# Autodesk Inventor assembly: Team_2374
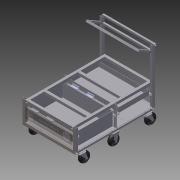
[picture p0: Inventor's stored thumbnail of the model, 180x180]
Saved by Autodesk Inventor 2012 (Build 160160000, 160)
## iProperties
Created: 2011-10-19
Part Number: Team_2374
Document SubType Name: Assembly
Designer: Ian Walters
Mass: 25411.4 g
Surface Area: 59424.9 cm^2
Volume: 9376.89 cm^3
Density: 2.71 g/cm^3
_SolveAssemblyDoc: Frame Generator Solve Assembly
_Version: 15.0.0
Author: Ian Walters
## Documents named in this file (38)
- C:\Users\Ian Walters\Dropbox\CAD Inventor\Preseason Projects\Cart Competition Cart\Team 2374\Team_2374.iam
- C:\Users\Ian Walters\Dropbox\CAD Inventor\Preseason Projects\Cart Competition Cart\Team 2374\Cart Skeleton.ipt
- C:\Users\Ian Walters\Dropbox\CAD Inventor\Preseason Projects\Cart Competition Cart\Team 2374\Team_2374\Frame\Cart Frame.iam
- C:\Users\Ian Walters\Dropbox\CAD Inventor\Preseason Projects\Cart Competition Cart\Team 2374\Bottom Sheet.ipt
- C:\Users\Ian Walters\Dropbox\CAD Inventor\Preseason Projects\Cart Competition Cart\Team 2374\IFI 114 - .1875 x 0.25.ipt
- C:\Users\Ian Walters\Dropbox\CAD Inventor\Preseason Projects\Cart Competition Cart\Team 2374\Fixed Caster.iam
- C:\Users\Ian Walters\Dropbox\CAD Inventor\Preseason Projects\Cart Competition Cart\Team 2374\Team_2374\Design Accelerator\Bolted Connection1.iam
- C:\Users\Ian Walters\Dropbox\CAD Inventor\Preseason Projects\Cart Competition Cart\Team 2374\Team_2374\Design Accelerator\Bolted Connection2.iam
- C:\Users\Ian Walters\Dropbox\CAD Inventor\Preseason Projects\Cart Competition Cart\Team 2374\Team_2374\Design Accelerator\Bolted Connection3.iam
- C:\Users\Ian Walters\Dropbox\CAD Inventor\Preseason Projects\Cart Competition Cart\Team 2374\Team_2374\Design Accelerator\Bolted Connection4.iam
- C:\Users\Ian Walters\Dropbox\CAD Inventor\Preseason Projects\Cart Competition Cart\Team 2374\Team_2374\Design Accelerator\Bolted Connection5.iam
- C:\Users\Ian Walters\Dropbox\CAD Inventor\Preseason Projects\Cart Competition Cart\Team 2374\Team_2374\Design Accelerator\Bolted Connection6.iam
- C:\Users\Ian Walters\Dropbox\CAD Inventor\Preseason Projects\Cart Competition Cart\Team 2374\Team_2374\Design Accelerator\Bolted Connection7.iam
- C:\Users\Ian Walters\Dropbox\CAD Inventor\Preseason Projects\Cart Competition Cart\Team 2374\Team_2374\Design Accelerator\Bolted Connection8.iam
- C:\Users\Ian Walters\Dropbox\CAD Inventor\Preseason Projects\Cart Competition Cart\Team 2374\Front Screen.ipt
- C:\Users\Ian Walters\Dropbox\CAD Inventor\Preseason Projects\Cart Competition Cart\Team 2374\Rotation Caster.iam
- C:\Users\Ian Walters\Dropbox\CAD Inventor\Preseason Projects\Cart Competition Cart\Team 2374\Team_2374\Design Accelerator\Bolted Connection9.iam
- C:\Users\Ian Walters\Dropbox\CAD Inventor\Preseason Projects\Cart Competition Cart\Team 2374\Team_2374\Design Accelerator\Bolted Connection10.iam
- C:\Users\Ian Walters\Dropbox\CAD Inventor\Preseason Projects\Cart Competition Cart\Team 2374\Team_2374\Design Accelerator\Bolted Connection11.iam
- C:\Users\Ian Walters\Dropbox\CAD Inventor\Preseason Projects\Cart Competition Cart\Team 2374\Team_2374\Design Accelerator\Bolted Connection12.iam
- C:\Users\Ian Walters\Dropbox\CAD Inventor\Preseason Projects\Cart Competition Cart\Team 2374\Team_2374\Design Accelerator\Bolted Connection13.iam
- C:\Users\Ian Walters\Dropbox\CAD Inventor\Preseason Projects\Cart Competition Cart\Team 2374\Team_2374\Design Accelerator\Bolted Connection14.iam
- C:\Users\Ian Walters\Dropbox\CAD Inventor\Preseason Projects\Cart Competition Cart\Team 2374\Team_2374\Design Accelerator\Bolted Connection15.iam
- C:\Users\Ian Walters\Dropbox\CAD Inventor\Preseason Projects\Cart Competition Cart\Team 2374\Team_2374\Design Accelerator\Bolted Connection16.iam
- C:\Users\Ian Walters\Dropbox\CAD Inventor\Preseason Projects\Cart Competition Cart\Team 2374\Team_2374\Design Accelerator\Bolted Connection17.iam
- C:\Users\Ian Walters\Dropbox\CAD Inventor\Preseason Projects\Cart Competition Cart\Team 2374\Team_2374\Design Accelerator\Bolted Connection18.iam
- C:\Users\Ian Walters\Dropbox\CAD Inventor\Preseason Projects\Cart Competition Cart\Team 2374\Team_2374\Design Accelerator\Bolted Connection19.iam
- C:\Users\Ian Walters\Dropbox\CAD Inventor\Preseason Projects\Cart Competition Cart\Team 2374\Team_2374\Design Accelerator\Bolted Connection20.iam
- C:\Users\Ian Walters\Dropbox\CAD Inventor\Preseason Projects\Cart Competition Cart\Team 2374\Team_2374\Design Accelerator\Bolted Connection21.iam
- C:\Users\Ian Walters\Dropbox\CAD Inventor\Preseason Projects\Cart Competition Cart\Team 2374\Team_2374\Design Accelerator\Bolted Connection22.iam
- C:\Users\Ian Walters\Dropbox\CAD Inventor\Preseason Projects\Cart Competition Cart\Team 2374\Team_2374\Design Accelerator\Bolted Connection23.iam
- C:\Users\Ian Walters\Dropbox\CAD Inventor\Preseason Projects\Cart Competition Cart\Team 2374\Team_2374\Design Accelerator\Bolted Connection24.iam
- C:\Users\Ian Walters\Dropbox\CAD Inventor\Preseason Projects\Cart Competition Cart\Team 2374\Drawer Slide.ipt
- C:\Users\Ian Walters\Dropbox\CAD Inventor\Preseason Projects\Cart Competition Cart\Team 2374\8020 Linear Bearing.iam
- C:\Users\Ian Walters\Dropbox\CAD Inventor\Preseason Projects\Cart Competition Cart\Team 2374\Big Drawer.ipt
- C:\Users\Ian Walters\Dropbox\CAD Inventor\Preseason Projects\Cart Competition Cart\Team 2374\Small Drawer.ipt
- C:\Users\Ian Walters\Dropbox\CAD Inventor\Preseason Projects\Cart Competition Cart\Team 2374\Handle.iam
- C:\Users\Ian Walters\Dropbox\CAD Inventor\Preseason Projects\Cart Competition Cart\Team 2374\Handle Slide.ipt
## Components (217 placed, 14 different names)
1. Cart Skeleton:1
2. Cart Frame:1 [sub-assembly] — Mate:1, Mate:2, Mate:3, Mate:4, Mate:5, Flush:1, Flush:2, Mate:26, Insert:11, Insert:12, Mate:29, Mate:30, Mate:31, Mate:32, Mate:33, Mate:34, Mate:35, Mate:36, Mate:37, Mate:38, Mate:39, Mate:40, Mate:41, Mate:42, Mate:43, Mate:44, Mate:45, Insert:13, Mate:46, Insert:14, Mate:47, Insert:15, Mate:48, Insert:16, Mate:49, Mate:50, Mate:51, Mate:52, Mate:53, Mate:54, Mate:55, Mate:56, Mate:57, Mate:58, Mate:59, Mate:60, Mate:61, Mate:62, Mate:63, Mate:64, Mate:65, Mate:66, Mate:67, Mate:68, Mate:69, Mate:70, Mate:71, Mate:72, Mate:73, Mate:74, Mate:75, Mate:76, Mate:77, Mate:78, Mate:79, Mate:80, Flush:3, Mate:81, Mate:83, Flush:21, Flush:22, Mate:92, Mate:93, Mate:94, Mate:95, Mate:96, Mate:99
3. Handle:1 [sub-assembly] — Mate:97, Mate:98, Mate:99
4. Handle Slide:2 — Mate:95, Mate:96, Flush:23
5. Handle Slide:1 — Mate:92, Mate:93, Mate:94, Flush:23, Mate:97, Mate:98
6. Bottom Sheet:1 — Mate:1, Mate:2, Mate:3, Insert:1, Insert:2, Insert:3, Insert:4, Mate:82
7. Front Screen:1 — Flush:1, Flush:2, Mate:26, Insert:7, Insert:8, Insert:9, Insert:10
8. Fixed Caster:1 [sub-assembly] — Mate:5, Insert:11
9. Fixed Caster:2 [sub-assembly] — Mate:4, Insert:12
10. Rotation Caster:1 [sub-assembly] — Mate:45, Insert:13
11. Rotation Caster:2 [sub-assembly] — Mate:46, Insert:14
12. Rotation Caster:3 [sub-assembly] — Mate:47, Insert:15
13. Rotation Caster:4 [sub-assembly] — Mate:48, Insert:16
14. IFI 114 - .1875 x 0.25:142 — Insert:10
15. IFI 114 - .1875 x 0.25:109 — Insert:7
16. Bolted Connection:1 [sub-assembly] — Mate:43, Mate:44
17. Bolted Connection:2 [sub-assembly] — Mate:29, Mate:30
18. Bolted Connection:3 [sub-assembly] — Mate:31, Mate:32
19. Bolted Connection:4 [sub-assembly] — Mate:33, Mate:34
20. Bolted Connection:5 [sub-assembly] — Mate:35, Mate:36
21. Bolted Connection:6 [sub-assembly] — Mate:37, Mate:38
22. Bolted Connection:7 [sub-assembly] — Mate:39, Mate:40
23. Bolted Connection:8 [sub-assembly] — Mate:41, Mate:42
24. Bolted Connection:9 [sub-assembly] — Mate:49, Mate:50
25. Bolted Connection:10 [sub-assembly] — Mate:51, Mate:52
26. Bolted Connection:11 [sub-assembly] — Mate:53, Mate:54
27. Bolted Connection:12 [sub-assembly] — Mate:55, Mate:56
28. Bolted Connection:13 [sub-assembly] — Mate:57, Mate:58
29. Bolted Connection:14 [sub-assembly] — Mate:59, Mate:60
30. Bolted Connection:15 [sub-assembly] — Mate:61, Mate:62
31. Bolted Connection:16 [sub-assembly] — Mate:63, Mate:64
32. Bolted Connection:17 [sub-assembly] — Mate:65, Mate:66
33. Bolted Connection:18 [sub-assembly] — Mate:67, Mate:68
34. Bolted Connection:19 [sub-assembly] — Mate:69, Mate:70
35. Bolted Connection:20 [sub-assembly] — Mate:71, Mate:72
36. Bolted Connection:21 [sub-assembly] — Mate:73, Mate:74
37. Bolted Connection:22 [sub-assembly] — Mate:75, Mate:76
38. Bolted Connection:23 [sub-assembly] — Mate:77, Mate:78
39. Bolted Connection:24 [sub-assembly] — Mate:79, Mate:80
40. Drawer Slide:1 — Flush:3, Mate:81, Mate:82, Flush:4, Flush:5, Flush:10, Flush:11, Flush:12, Flush:13
41. Drawer Slide:2 — Flush:4, Flush:5, Flush:9, Flush:16, Flush:17, Flush:18, Flush:19, Mate:89, Flush:8
42. Drawer Slide:3 — Flush:6, Flush:7, Flush:9, Mate:83, Mate:86, Flush:20, Mate:87, Mate:88
43. Drawer Slide:4 — Flush:6, Flush:7, Flush:8, Mate:84, Flush:14, Mate:85, Flush:15, Mate:89
44. 8020 Linear Bearing:1 [sub-assembly] — Flush:12, Flush:13, Insert:17, Insert:18
45. 8020 Linear Bearing:2 [sub-assembly] — Flush:10, Flush:11, Insert:19
46. 8020 Linear Bearing:3 [sub-assembly] — Mate:84, Flush:14, Insert:21
47. 8020 Linear Bearing:4 [sub-assembly] — Mate:85, Flush:15, Insert:20
48. 8020 Linear Bearing:5 [sub-assembly] — Flush:16, Flush:17, Mate:90
49. 8020 Linear Bearing:6 [sub-assembly] — Flush:18, Flush:19, Mate:91
50. 8020 Linear Bearing:7 [sub-assembly] — Mate:86, Flush:20, Insert:24
51. 8020 Linear Bearing:8 [sub-assembly] — Mate:87, Mate:88, Insert:22, Insert:23
52. Big Drawer:1 — Insert:17, Insert:18, Insert:19, Insert:20, Insert:21, Flush:21
53. Small Drawer:1 — Insert:22, Insert:23, Insert:24, Mate:90, Mate:91, Flush:22
54. IFI 114 - .1875 x 0.25:1 — Insert:1
55. IFI 114 - .1875 x 0.25:2 — Insert:2
56. IFI 114 - .1875 x 0.25:3 — Insert:3
57. IFI 114 - .1875 x 0.25:4 — Insert:4
58. IFI 114 - .1875 x 0.25:5
59. IFI 114 - .1875 x 0.25:6
60. IFI 114 - .1875 x 0.25:7
61. IFI 114 - .1875 x 0.25:8
62. IFI 114 - .1875 x 0.25:9
63. IFI 114 - .1875 x 0.25:10
64. IFI 114 - .1875 x 0.25:11
65. IFI 114 - .1875 x 0.25:12
66. IFI 114 - .1875 x 0.25:13
67. IFI 114 - .1875 x 0.25:14
68. IFI 114 - .1875 x 0.25:15
69. IFI 114 - .1875 x 0.25:16
70. IFI 114 - .1875 x 0.25:17
71. IFI 114 - .1875 x 0.25:18
72. IFI 114 - .1875 x 0.25:19
73. IFI 114 - .1875 x 0.25:20
74. IFI 114 - .1875 x 0.25:21
75. IFI 114 - .1875 x 0.25:22
76. IFI 114 - .1875 x 0.25:23
77. IFI 114 - .1875 x 0.25:24
78. IFI 114 - .1875 x 0.25:25
79. IFI 114 - .1875 x 0.25:26
80. IFI 114 - .1875 x 0.25:27
81. IFI 114 - .1875 x 0.25:28
82. IFI 114 - .1875 x 0.25:29
83. IFI 114 - .1875 x 0.25:30
84. IFI 114 - .1875 x 0.25:31
85. IFI 114 - .1875 x 0.25:32
86. IFI 114 - .1875 x 0.25:33
87. IFI 114 - .1875 x 0.25:34
88. IFI 114 - .1875 x 0.25:35
89. IFI 114 - .1875 x 0.25:36
90. IFI 114 - .1875 x 0.25:37
91. IFI 114 - .1875 x 0.25:38
92. IFI 114 - .1875 x 0.25:39
93. IFI 114 - .1875 x 0.25:40
94. IFI 114 - .1875 x 0.25:41
95. IFI 114 - .1875 x 0.25:42
96. IFI 114 - .1875 x 0.25:43
97. IFI 114 - .1875 x 0.25:44
98. IFI 114 - .1875 x 0.25:45
99. IFI 114 - .1875 x 0.25:46
100. IFI 114 - .1875 x 0.25:47
101. IFI 114 - .1875 x 0.25:48
102. IFI 114 - .1875 x 0.25:49
103. IFI 114 - .1875 x 0.25:50
104. IFI 114 - .1875 x 0.25:51
105. IFI 114 - .1875 x 0.25:52
106. IFI 114 - .1875 x 0.25:53
107. IFI 114 - .1875 x 0.25:54
108. IFI 114 - .1875 x 0.25:55
109. IFI 114 - .1875 x 0.25:56
110. IFI 114 - .1875 x 0.25:57
111. IFI 114 - .1875 x 0.25:58
112. IFI 114 - .1875 x 0.25:59
113. IFI 114 - .1875 x 0.25:60
114. IFI 114 - .1875 x 0.25:61
115. IFI 114 - .1875 x 0.25:62
116. IFI 114 - .1875 x 0.25:63
117. IFI 114 - .1875 x 0.25:64
118. IFI 114 - .1875 x 0.25:65
119. IFI 114 - .1875 x 0.25:66
120. IFI 114 - .1875 x 0.25:67
121. IFI 114 - .1875 x 0.25:68
122. IFI 114 - .1875 x 0.25:69
123. IFI 114 - .1875 x 0.25:70
124. IFI 114 - .1875 x 0.25:71
125. IFI 114 - .1875 x 0.25:72
126. IFI 114 - .1875 x 0.25:73
127. IFI 114 - .1875 x 0.25:74
128. IFI 114 - .1875 x 0.25:75
129. IFI 114 - .1875 x 0.25:76
130. IFI 114 - .1875 x 0.25:77
131. IFI 114 - .1875 x 0.25:78
132. IFI 114 - .1875 x 0.25:79
133. IFI 114 - .1875 x 0.25:80
134. IFI 114 - .1875 x 0.25:81
135. IFI 114 - .1875 x 0.25:82
136. IFI 114 - .1875 x 0.25:83
137. IFI 114 - .1875 x 0.25:84
138. IFI 114 - .1875 x 0.25:85
139. IFI 114 - .1875 x 0.25:86
140. IFI 114 - .1875 x 0.25:87
141. IFI 114 - .1875 x 0.25:88
142. IFI 114 - .1875 x 0.25:89
143. IFI 114 - .1875 x 0.25:90
144. IFI 114 - .1875 x 0.25:91
145. IFI 114 - .1875 x 0.25:92
146. IFI 114 - .1875 x 0.25:93
147. IFI 114 - .1875 x 0.25:94
148. IFI 114 - .1875 x 0.25:95
149. IFI 114 - .1875 x 0.25:96
150. IFI 114 - .1875 x 0.25:97
151. IFI 114 - .1875 x 0.25:98
152. IFI 114 - .1875 x 0.25:99
153. IFI 114 - .1875 x 0.25:100
154. IFI 114 - .1875 x 0.25:101
155. IFI 114 - .1875 x 0.25:102
156. IFI 114 - .1875 x 0.25:103
157. IFI 114 - .1875 x 0.25:104
158. IFI 114 - .1875 x 0.25:105
159. IFI 114 - .1875 x 0.25:106
160. IFI 114 - .1875 x 0.25:107
161. IFI 114 - .1875 x 0.25:108
162. IFI 114 - .1875 x 0.25:110 — Insert:8
163. IFI 114 - .1875 x 0.25:111
164. IFI 114 - .1875 x 0.25:112
165. IFI 114 - .1875 x 0.25:113
166. IFI 114 - .1875 x 0.25:114
167. IFI 114 - .1875 x 0.25:115
168. IFI 114 - .1875 x 0.25:116
169. IFI 114 - .1875 x 0.25:117
170. IFI 114 - .1875 x 0.25:118
171. IFI 114 - .1875 x 0.25:119
172. IFI 114 - .1875 x 0.25:120
173. IFI 114 - .1875 x 0.25:121
174. IFI 114 - .1875 x 0.25:122
175. IFI 114 - .1875 x 0.25:123
176. IFI 114 - .1875 x 0.25:124
177. IFI 114 - .1875 x 0.25:125
178. IFI 114 - .1875 x 0.25:126
179. IFI 114 - .1875 x 0.25:127
180. IFI 114 - .1875 x 0.25:128
181. IFI 114 - .1875 x 0.25:129
182. IFI 114 - .1875 x 0.25:130
183. IFI 114 - .1875 x 0.25:131
184. IFI 114 - .1875 x 0.25:132
185. IFI 114 - .1875 x 0.25:133
186. IFI 114 - .1875 x 0.25:134
187. IFI 114 - .1875 x 0.25:135
188. IFI 114 - .1875 x 0.25:136
189. IFI 114 - .1875 x 0.25:137
190. IFI 114 - .1875 x 0.25:138
191. IFI 114 - .1875 x 0.25:139
192. IFI 114 - .1875 x 0.25:140
193. IFI 114 - .1875 x 0.25:141 — Insert:9
194. IFI 114 - .1875 x 0.25:143
195. IFI 114 - .1875 x 0.25:144
196. IFI 114 - .1875 x 0.25:145
197. IFI 114 - .1875 x 0.25:146
198. IFI 114 - .1875 x 0.25:147
199. IFI 114 - .1875 x 0.25:148
200. IFI 114 - .1875 x 0.25:149
201. IFI 114 - .1875 x 0.25:150
202. IFI 114 - .1875 x 0.25:151
203. IFI 114 - .1875 x 0.25:152
204. IFI 114 - .1875 x 0.25:153
205. IFI 114 - .1875 x 0.25:154
206. IFI 114 - .1875 x 0.25:155
207. IFI 114 - .1875 x 0.25:156
208. IFI 114 - .1875 x 0.25:157
209. IFI 114 - .1875 x 0.25:158
210. IFI 114 - .1875 x 0.25:159
211. IFI 114 - .1875 x 0.25:160
212. IFI 114 - .1875 x 0.25:161
213. IFI 114 - .1875 x 0.25:162
214. IFI 114 - .1875 x 0.25:163
215. IFI 114 - .1875 x 0.25:164
216. IFI 114 - .1875 x 0.25:165
217. IFI 114 - .1875 x 0.25:166
## Component patterns: (27 elements, first: IFI 114 - .1875 x 0.25:1 + IFI 114 - .1875 x 0.25:2 + IFI 114 - .1875 x 0.25:3 + IFI 114 - .1875 x 0.25:4), (31 elements, first: IFI 114 - .1875 x 0.25:110), (25 elements, first: IFI 114 - .1875 x 0.25:141)
## Relationships (122: Mate 77, Flush 23, Insert 22)
- Mate:1: Cart Frame:1 ↔ Bottom Sheet:1
- Mate:2: Cart Frame:1 ↔ Bottom Sheet:1
- Mate:3: Cart Frame:1 ↔ Bottom Sheet:1
- Insert:1: Bottom Sheet:1 ↔ IFI 114 - .1875 x 0.25:1
- Insert:2: Bottom Sheet:1 ↔ IFI 114 - .1875 x 0.25:2
- Insert:3: Bottom Sheet:1 ↔ IFI 114 - .1875 x 0.25:3
- Insert:4: Bottom Sheet:1 ↔ IFI 114 - .1875 x 0.25:4
- Mate:4: Cart Frame:1 ↔ Fixed Caster:2
- Mate:5: Cart Frame:1 ↔ Fixed Caster:1
- Flush:1: Cart Frame:1 ↔ Front Screen:1
- Flush:2: Cart Frame:1 ↔ Front Screen:1
- Mate:26: Cart Frame:1 ↔ Front Screen:1
- Insert:7: Front Screen:1 ↔ IFI 114 - .1875 x 0.25:109
- Insert:8: Front Screen:1 ↔ IFI 114 - .1875 x 0.25:110
- Insert:9: Front Screen:1 ↔ IFI 114 - .1875 x 0.25:141
- Insert:10: Front Screen:1 ↔ IFI 114 - .1875 x 0.25:142
- Insert:11: Cart Frame:1 ↔ Fixed Caster:1
- Insert:12: Cart Frame:1 ↔ Fixed Caster:2
- Mate:29: Cart Frame:1 ↔ Bolted Connection:2
- Mate:30: Cart Frame:1 ↔ Bolted Connection:2
- Mate:31: Cart Frame:1 ↔ Bolted Connection:3
- Mate:32: Cart Frame:1 ↔ Bolted Connection:3
- Mate:33: Cart Frame:1 ↔ Bolted Connection:4
- Mate:34: Cart Frame:1 ↔ Bolted Connection:4
- Mate:35: Cart Frame:1 ↔ Bolted Connection:5
- Mate:36: Cart Frame:1 ↔ Bolted Connection:5
- Mate:37: Cart Frame:1 ↔ Bolted Connection:6
- Mate:38: Cart Frame:1 ↔ Bolted Connection:6
- Mate:39: Cart Frame:1 ↔ Bolted Connection:7
- Mate:40: Cart Frame:1 ↔ Bolted Connection:7
- Mate:41: Cart Frame:1 ↔ Bolted Connection:8
- Mate:42: Cart Frame:1 ↔ Bolted Connection:8
- Mate:43: Cart Frame:1 ↔ Bolted Connection:1
- Mate:44: Cart Frame:1 ↔ Bolted Connection:1
- Mate:45: Cart Frame:1 ↔ Rotation Caster:1
- Insert:13: Cart Frame:1 ↔ Rotation Caster:1
- Mate:46: Cart Frame:1 ↔ Rotation Caster:2
- Insert:14: Cart Frame:1 ↔ Rotation Caster:2
- Mate:47: Cart Frame:1 ↔ Rotation Caster:3
- Insert:15: Cart Frame:1 ↔ Rotation Caster:3
- Mate:48: Cart Frame:1 ↔ Rotation Caster:4
- Insert:16: Cart Frame:1 ↔ Rotation Caster:4
- Mate:49: Cart Frame:1 ↔ Bolted Connection:9
- Mate:50: Cart Frame:1 ↔ Bolted Connection:9
- Mate:51: Cart Frame:1 ↔ Bolted Connection:10
- Mate:52: Cart Frame:1 ↔ Bolted Connection:10
- Mate:53: Cart Frame:1 ↔ Bolted Connection:11
- Mate:54: Cart Frame:1 ↔ Bolted Connection:11
- Mate:55: Cart Frame:1 ↔ Bolted Connection:12
- Mate:56: Cart Frame:1 ↔ Bolted Connection:12
- Mate:57: Cart Frame:1 ↔ Bolted Connection:13
- Mate:58: Cart Frame:1 ↔ Bolted Connection:13
- Mate:59: Cart Frame:1 ↔ Bolted Connection:14
- Mate:60: Cart Frame:1 ↔ Bolted Connection:14
- Mate:61: Cart Frame:1 ↔ Bolted Connection:15
- Mate:62: Cart Frame:1 ↔ Bolted Connection:15
- Mate:63: Cart Frame:1 ↔ Bolted Connection:16
- Mate:64: Cart Frame:1 ↔ Bolted Connection:16
- Mate:65: Cart Frame:1 ↔ Bolted Connection:17
- Mate:66: Cart Frame:1 ↔ Bolted Connection:17
- Mate:67: Cart Frame:1 ↔ Bolted Connection:18
- Mate:68: Cart Frame:1 ↔ Bolted Connection:18
- Mate:69: Cart Frame:1 ↔ Bolted Connection:19
- Mate:70: Cart Frame:1 ↔ Bolted Connection:19
- Mate:71: Cart Frame:1 ↔ Bolted Connection:20
- Mate:72: Cart Frame:1 ↔ Bolted Connection:20
- Mate:73: Cart Frame:1 ↔ Bolted Connection:21
- Mate:74: Cart Frame:1 ↔ Bolted Connection:21
- Mate:75: Cart Frame:1 ↔ Bolted Connection:22
- Mate:76: Cart Frame:1 ↔ Bolted Connection:22
- Mate:77: Cart Frame:1 ↔ Bolted Connection:23
- Mate:78: Cart Frame:1 ↔ Bolted Connection:23
- Mate:79: Cart Frame:1 ↔ Bolted Connection:24
- Mate:80: Cart Frame:1 ↔ Bolted Connection:24
- Flush:3: Cart Frame:1 ↔ Drawer Slide:1
- Mate:81: Cart Frame:1 ↔ Drawer Slide:1
- Mate:82 (152.4 mm): Bottom Sheet:1 ↔ Drawer Slide:1
- Flush:4: Drawer Slide:1 ↔ Drawer Slide:2
- Flush:5: Drawer Slide:1 ↔ Drawer Slide:2
- Flush:6: Drawer Slide:3 ↔ Drawer Slide:4
- Flush:7: Drawer Slide:3 ↔ Drawer Slide:4
- Flush:8: Drawer Slide:2 ↔ Drawer Slide:4
- Flush:9: Drawer Slide:2 ↔ Drawer Slide:3
- Mate:83: Cart Frame:1 ↔ Drawer Slide:3
- Flush:10: Drawer Slide:1 ↔ 8020 Linear Bearing:2
- Flush:11: Drawer Slide:1 ↔ 8020 Linear Bearing:2
- Flush:12: Drawer Slide:1 ↔ 8020 Linear Bearing:1
- Flush:13: Drawer Slide:1 ↔ 8020 Linear Bearing:1
- Mate:84: Drawer Slide:4 ↔ 8020 Linear Bearing:3
- Flush:14: Drawer Slide:4 ↔ 8020 Linear Bearing:3
- Mate:85: Drawer Slide:4 ↔ 8020 Linear Bearing:4
- Flush:15: Drawer Slide:4 ↔ 8020 Linear Bearing:4
- Flush:16: Drawer Slide:2 ↔ 8020 Linear Bearing:5
- Flush:17: Drawer Slide:2 ↔ 8020 Linear Bearing:5
- Flush:18: Drawer Slide:2 ↔ 8020 Linear Bearing:6
- Flush:19: Drawer Slide:2 ↔ 8020 Linear Bearing:6
- Mate:86: Drawer Slide:3 ↔ 8020 Linear Bearing:7
- Flush:20: Drawer Slide:3 ↔ 8020 Linear Bearing:7
- Mate:87: Drawer Slide:3 ↔ 8020 Linear Bearing:8
- Mate:88: Drawer Slide:3 ↔ 8020 Linear Bearing:8
- Insert:17: 8020 Linear Bearing:1 ↔ Big Drawer:1
- Insert:18: 8020 Linear Bearing:1 ↔ Big Drawer:1
- Insert:19: 8020 Linear Bearing:2 ↔ Big Drawer:1
- Insert:20: 8020 Linear Bearing:4 ↔ Big Drawer:1
- Insert:21: 8020 Linear Bearing:3 ↔ Big Drawer:1
- Flush:21: Cart Frame:1 ↔ Big Drawer:1
- Mate:89 (25.4 mm): Drawer Slide:2 ↔ Drawer Slide:4
- Insert:22: 8020 Linear Bearing:8 ↔ Small Drawer:1
- Insert:23: 8020 Linear Bearing:8 ↔ Small Drawer:1
- Insert:24: 8020 Linear Bearing:7 ↔ Small Drawer:1
- Mate:90: 8020 Linear Bearing:5 ↔ Small Drawer:1
- Mate:91: 8020 Linear Bearing:6 ↔ Small Drawer:1
- Flush:22: Cart Frame:1 ↔ Small Drawer:1
- Mate:92: Cart Frame:1 ↔ Handle Slide:1
- Mate:93: Cart Frame:1 ↔ Handle Slide:1
- Mate:94 (101.6 mm): Cart Frame:1 ↔ Handle Slide:1
- Mate:95: Cart Frame:1 ↔ Handle Slide:2
- Mate:96: Cart Frame:1 ↔ Handle Slide:2
- Flush:23: Handle Slide:2 ↔ Handle Slide:1
- Mate:97: Handle:1 ↔ Handle Slide:1
- Mate:98: Handle:1 ↔ Handle Slide:1
- Mate:99: Cart Frame:1 ↔ Handle:1
